# Autodesk Inventor assembly: bett_V2_klappe
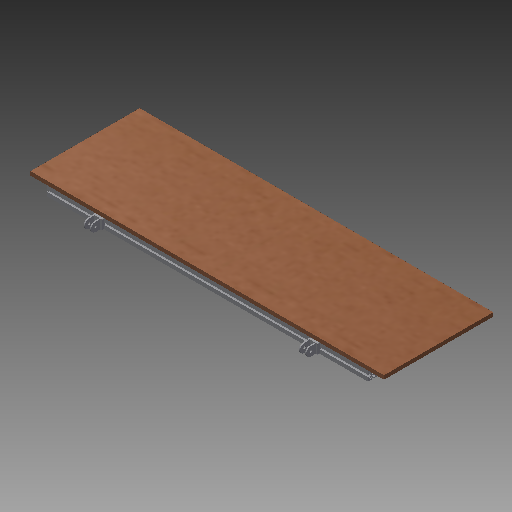
[picture p0: Inventor's stored thumbnail of the model, 512x512]
Saved by Autodesk Inventor 2018 (Build 220112000, 112)
## iProperties
Created: 2020-03-29
Part Number: bett_V2_klappe
Material: Generisch
Document SubType Name: Assembly
Designer: wepet
Author: wepet
## Documents named in this file (7)
- C:\Users\wepet\Downloads\anhaenger\current\details\bett\bett_V2\bett_V2_teil3_klappe.iam
- C:\Users\wepet\Downloads\anhaenger\current\details\bett\details\item_winkel.ipt
- C:\Users\wepet\Downloads\anhaenger\current\details\bett\details\item_gelenk_teil_quer.ipt
- C:\Users\wepet\Downloads\anhaenger\current\details\bett\details\item_30x30_25cm.ipt
- C:\Users\wepet\Downloads\anhaenger\current\details\bett\bett_V2\bett_V2_detail_deckplatte_klappe.ipt
- C:\Users\wepet\Downloads\anhaenger\current\details\bett\details\item_30x30_100cm.ipt
- C:\Users\wepet\Downloads\anhaenger\current\details\bett\details\item_scharnier_1_teil.ipt
## Components (13 placed, 6 different names)
1. item_30x30_100cm:1 — Fluchtend:11, Fluchtend:16, Passend:8, Fluchtend:23, Passend:31, Fluchtend:122, Passend:66, Passend:71, Passend:72, Fluchtend:197, Fluchtend:198, Passend:73, Passend:74, Fluchtend:201, Fluchtend:202, Fluchtend:203, Passend:76, Passend:79, Fluchtend:209
2. item_30x30_100cm:2 — Fluchtend:11, Fluchtend:24, Fluchtend:82, Passend:69, Fluchtend:204, Passend:75, Passend:78, Passend:80, Passend:81, Fluchtend:207, Fluchtend:208
3. item_30x30_25cm:1 — Fluchtend:16, Passend:8, Fluchtend:203, Fluchtend:204, Passend:75, Passend:77, Passend:83
4. item_30x30_25cm:2 — Fluchtend:23, Fluchtend:24, Passend:29, Fluchtend:196, Fluchtend:200, Passend:76, Fluchtend:206, Passend:82
5. item_winkel:19 — Passend:29, Passend:31, Fluchtend:196
6. item_winkel:20 — Fluchtend:82, Passend:69
7. item_winkel:25 — Passend:77, Passend:78
8. item_winkel:26 — Fluchtend:122, Passend:66
9. item_gelenk_teil_quer:1 — Passend:71, Fluchtend:198, Fluchtend:200
10. item_gelenk_teil_quer:2 — Passend:72, Fluchtend:197, Fluchtend:202
11. bett_V2_detail_deckplatte_klappe:1 — Passend:79, Fluchtend:206, Fluchtend:209
12. item_scharnier_1_teil:1 — Passend:80, Fluchtend:207, Passend:82
13. item_scharnier_1_teil:2 — Passend:81, Fluchtend:208, Passend:83
## Relationships (40: Flush 22, Mate 18)
- Fluchtend:11 [Flush]: item_30x30_100cm:1 ↔ item_30x30_100cm:2
- Fluchtend:16 [Flush]: item_30x30_100cm:1 ↔ item_30x30_25cm:1
- Passend:8 [Mate]: item_30x30_100cm:1 ↔ item_30x30_25cm:1
- Fluchtend:23 [Flush]: item_30x30_100cm:1 ↔ item_30x30_25cm:2
- Fluchtend:24 [Flush]: item_30x30_100cm:2 ↔ item_30x30_25cm:2
- [Flush]: item_winkel:19 ↔ item_winkel:20
- Passend:29 [Mate]: item_30x30_25cm:2 ↔ item_winkel:19
- Passend:31 [Mate]: item_30x30_100cm:1 ↔ item_winkel:19
- Fluchtend:82 [Flush]: item_30x30_100cm:2 ↔ item_winkel:20
- [Flush]: item_winkel:25 ↔ item_winkel:26
- [Flush]: item_winkel:25 ↔ item_winkel:26
- [Flush]: item_winkel:25 ↔ item_winkel:26
- Fluchtend:122 [Flush]: item_30x30_100cm:1 ↔ item_winkel:26
- Passend:66 [Mate]: item_30x30_100cm:1 ↔ item_winkel:26
- Passend:69 [Mate]: item_30x30_100cm:2 ↔ item_winkel:20
- Fluchtend:196 [Flush]: item_30x30_25cm:2 ↔ item_winkel:19
- Passend:71 [Mate]: item_30x30_100cm:1 ↔ item_gelenk_teil_quer:1
- Passend:72 [Mate]: item_30x30_100cm:1 ↔ item_gelenk_teil_quer:2
- Fluchtend:197 [Flush]: item_30x30_100cm:1 ↔ item_gelenk_teil_quer:2
- Fluchtend:198 [Flush]: item_30x30_100cm:1 ↔ item_gelenk_teil_quer:1
- Fluchtend:200 [Flush] (15 mm): item_30x30_25cm:2 ↔ item_gelenk_teil_quer:1
- Passend:73 [Mate]: item_30x30_100cm:1
- Passend:74 [Mate]: item_30x30_100cm:1
- Fluchtend:201 [Flush]: item_30x30_100cm:1
- Fluchtend:202 [Flush] (15 mm): item_30x30_100cm:1 ↔ item_gelenk_teil_quer:2
- Fluchtend:203 [Flush]: item_30x30_100cm:1 ↔ item_30x30_25cm:1
- Fluchtend:204 [Flush]: item_30x30_100cm:2 ↔ item_30x30_25cm:1
- Passend:75 [Mate]: item_30x30_100cm:2 ↔ item_30x30_25cm:1
- Passend:76 [Mate]: item_30x30_100cm:1 ↔ item_30x30_25cm:2
- Passend:77 [Mate]: item_30x30_25cm:1 ↔ item_winkel:25
- Passend:78 [Mate]: item_30x30_100cm:2 ↔ item_winkel:25
- Passend:79 [Mate]: item_30x30_100cm:1 ↔ bett_V2_detail_deckplatte_klappe:1
- Fluchtend:206 [Flush] (-5 mm): item_30x30_25cm:2 ↔ bett_V2_detail_deckplatte_klappe:1
- Passend:80 [Mate]: item_30x30_100cm:2 ↔ item_scharnier_1_teil:1
- Passend:81 [Mate]: item_30x30_100cm:2 ↔ item_scharnier_1_teil:2
- Fluchtend:207 [Flush] (-0.5 mm): item_30x30_100cm:2 ↔ item_scharnier_1_teil:1
- Fluchtend:208 [Flush] (0.5 mm): item_30x30_100cm:2 ↔ item_scharnier_1_teil:2
- Passend:82 [Mate] (-6.9 mm): item_30x30_25cm:2 ↔ item_scharnier_1_teil:1
- Passend:83 [Mate] (-6.9 mm): item_30x30_25cm:1 ↔ item_scharnier_1_teil:2
- Fluchtend:209 [Flush]: item_30x30_100cm:1 ↔ bett_V2_detail_deckplatte_klappe:1
## Named parameters: d113_d68 = 0 mm, d136_d106_d61_d60 = 0 mm, d139_d109_d64 = 0 mm, d145_d115_d70 = 0 mm
